# Autodesk Inventor assembly: TENSIONER
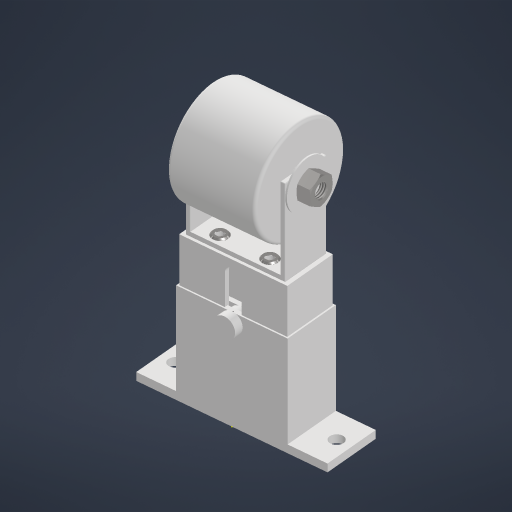
[picture p0: Inventor's stored thumbnail of the model, 512x512]
Saved by Autodesk Inventor 2023 (Build 270158000, 158)
## iProperties
Created: 2023-12-28
Part Number: TENSIONER
Document SubType Name: Assembly
Designer: User
Author: User
## Documents named in this file (12)
- C:\Users\User\Desktop\PROJECTS\CHAIN AND BELT SYSTEM\TENSIONER.iam
- C:\Users\User\Desktop\PROJECTS\CHAIN AND BELT SYSTEM\BEARING.ipt
- C:\Users\User\Desktop\PROJECTS\CHAIN AND BELT SYSTEM\HOLDER.ipt
- C:\Users\User\Desktop\PROJECTS\CHAIN AND BELT SYSTEM\ROLLER.ipt
- C:\Users\User\Desktop\PROJECTS\CHAIN AND BELT SYSTEM\WASHER.ipt
- C:\Users\User\Desktop\PROJECTS\CHAIN AND BELT SYSTEM\ROLLER SHAFT.ipt
- C:\Users\User\Documents\Inventor\Content Center Files\R2023\en-US\ANSI B 18.2.4.1 M(1)\ANSI B 18.2.4.1 M - M10 x 1.5Style 1.ipt
- C:\Users\User\Desktop\PROJECTS\CHAIN AND BELT SYSTEM\SLIDER.ipt
- C:\Users\User\Documents\Inventor\Content Center Files\R2023\en-US\ANSI B18.3.6M(07)\ANSI B18.3.6M - M10x1.5 x 8(7).ipt
- C:\Users\User\Desktop\PROJECTS\CHAIN AND BELT SYSTEM\BOTTOM STOPPER.ipt
- C:\Users\User\Desktop\PROJECTS\CHAIN AND BELT SYSTEM\BASE.ipt
- C:\Users\User\Desktop\PROJECTS\CHAIN AND BELT SYSTEM\TOP STOPPER.ipt
## Components (17 placed, 11 different names)
1. HOLDER:1 — Insert:3, Insert:4, Rotation:6, Rigid:1, Rigid:2, Rigid:3, Rigid:4, Rigid:5, Insert:10
2. ROLLER:1 — Insert:1, Insert:2
3. WASHER:1 — Insert:3, Insert:8
4. WASHER:2 — Insert:4, Insert:6, Insert:9
5. BEARING:1 — Insert:2, Rotation:6
6. BEARING:2 — Insert:1, Insert:10
7. ROLLER SHAFT:1 — Insert:6
8. Hex Nut Metric M10 x 1.5:1 — Insert:9
9. Hex Nut Metric M10 x 1.5:2 — Insert:8
10. SLIDER:1 — Rigid:1, Flush:1, Mate:1
11. Forged Hexagon Socket Set Screw - Oval Point - Metric M10x1.5 x 8:1 — Rigid:2
12. Forged Hexagon Socket Set Screw - Oval Point - Metric M10x1.5 x 8:2 — Rigid:5
13. Forged Hexagon Socket Set Screw - Oval Point - Metric M10x1.5 x 8:3 — Rigid:3
14. Forged Hexagon Socket Set Screw - Oval Point - Metric M10x1.5 x 8:4 — Rigid:4
15. BOTTOM STOPPER:1 — Rigid:6, Rigid:7
16. BASE:1 — Flush:1, Mate:1, Rigid:6
17. TOP STOPPER:1 — Rigid:7
## Relationships (18: Insert 8, WeldJoint 7, RelateRotation 1, Flush 1, Mate 1)
- Insert:1 (-10 mm): ROLLER:1 ↔ BEARING:2
- Insert:2 (-10 mm): ROLLER:1 ↔ BEARING:1
- Insert:3: HOLDER:1 ↔ WASHER:1
- Insert:4: HOLDER:1 ↔ WASHER:2
- Rotation:6 [RelateRotation] (1 ul): HOLDER:1 ↔ BEARING:1
- Insert:6 (-66 mm): WASHER:2 ↔ ROLLER SHAFT:1
- Insert:8: WASHER:1 ↔ Hex Nut Metric M10 x 1.5:2
- Insert:9: WASHER:2 ↔ Hex Nut Metric M10 x 1.5:1
- Rigid:1 [WeldJoint]: HOLDER:1 ↔ SLIDER:1
- Rigid:2 [WeldJoint]: HOLDER:1 ↔ Forged Hexagon Socket Set Screw - Oval Point - Metric M10x1.5 x 8:1
- Rigid:3 [WeldJoint]: HOLDER:1 ↔ Forged Hexagon Socket Set Screw - Oval Point - Metric M10x1.5 x 8:3
- Rigid:4 [WeldJoint]: HOLDER:1 ↔ Forged Hexagon Socket Set Screw - Oval Point - Metric M10x1.5 x 8:4
- Rigid:5 [WeldJoint]: HOLDER:1 ↔ Forged Hexagon Socket Set Screw - Oval Point - Metric M10x1.5 x 8:2
- Insert:10 (0.5 mm): HOLDER:1 ↔ BEARING:2
- Flush:1: SLIDER:1 ↔ BASE:1
- Mate:1: SLIDER:1 ↔ BASE:1
- Rigid:6 [WeldJoint] (-6 mm): BOTTOM STOPPER:1 ↔ BASE:1
- Rigid:7 [WeldJoint]: BOTTOM STOPPER:1 ↔ TOP STOPPER:1
